# Autodesk Inventor assembly: Arm Assembly
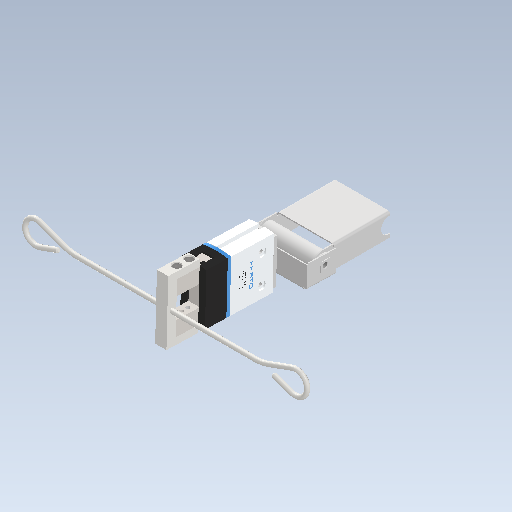
[picture p0: Inventor's stored thumbnail of the model, 512x512]
Saved by Autodesk Inventor 2021 (Build 250183000, 183)
## iProperties
Created: 2020-11-04
Part Number: Arm Assembly
Document SubType Name: Assembly
Designer: Alfred Brauner
Author: Alfred Brauner
## Documents named in this file (7)
- C:\Users\soeren\Downloads\STOMPA\STOMPA\Arm Assembly.iam
- C:\Users\soeren\Downloads\STOMPA\STOMPA\Joint0_Joint1_Link.ipt
- C:\Users\soeren\Downloads\STOMPA\STOMPA\Arm o14 bushing.ipt
- C:\Users\soeren\Downloads\STOMPA\STOMPA\Joint1_Shaft.ipt
- C:\Users\soeren\Downloads\STOMPA\STOMPA\Joint1_Bracket.ipt
- C:\Users\soeren\Downloads\STOMPA\STOMPA\90 graders beslag.ipt
- C:\Users\soeren\Downloads\STOMPA\STOMPA\Montagem da garra festo.iam
## Components (6 placed, 6 different names)
1. arm 1 v2:1 — Mate:1, Flush:1
2. Arm o14 bushing:1 — Mate:1, Flush:1, Mate:11, Flush:4
3. Revolver shaft:1 — Mate:11, Flush:4, Mate:12, Mate:13, Mate:14
4. Arm bracket:1 — Mate:6, Mate:7, Flush:3, Mate:12, Mate:13, Mate:14
5. 90 graders beslag:1 — Mate:6, Mate:7, Flush:3, Mate:8, Mate:9, Mate:10
6. Montagem da garra festo:1 [sub-assembly] — Mate:8, Mate:9, Mate:10
## Relationships (13: Mate 10, Flush 3)
- Mate:1: arm 1 v2:1 ↔ Arm o14 bushing:1
- Flush:1 (-1 mm): arm 1 v2:1 ↔ Arm o14 bushing:1
- Mate:6: Arm bracket:1 ↔ 90 graders beslag:1
- Mate:7 (-29.5 mm): Arm bracket:1 ↔ 90 graders beslag:1
- Flush:3 (-6.75 mm): Arm bracket:1 ↔ 90 graders beslag:1
- Mate:8: 90 graders beslag:1 ↔ Montagem da garra festo:1
- Mate:9: 90 graders beslag:1 ↔ Montagem da garra festo:1
- Mate:10: 90 graders beslag:1 ↔ Montagem da garra festo:1
- Mate:11: Arm o14 bushing:1 ↔ Revolver shaft:1
- Flush:4 (-0.25 mm): Arm o14 bushing:1 ↔ Revolver shaft:1
- Mate:12: Revolver shaft:1 ↔ Arm bracket:1
- Mate:13: Revolver shaft:1 ↔ Arm bracket:1
- Mate:14: Revolver shaft:1 ↔ Arm bracket:1
